# Autodesk Inventor assembly: ploter
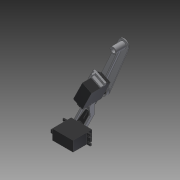
[picture p0: Inventor's stored thumbnail of the model, 180x180]
Saved by Autodesk Inventor 2013 (Build 170138000, 138)
## iProperties
Created: 2013-03-06
Part Number: ploter
Document SubType Name: Assembly
Designer: Masta
Author: Masta
## Documents named in this file (6)
- D:\work\ploter trapezowy arduino\ploter.iam
- D:\work\ploter trapezowy arduino\serwo HX12K.ipt
- D:\work\ploter trapezowy arduino\orczyk do HS12K duzy jednostronny.ipt
- D:\work\ploter trapezowy arduino\ramie1.ipt
- D:\work\ploter trapezowy arduino\ramie2.ipt
- D:\work\ploter trapezowy arduino\orczyk do SRM-102 okragly.ipt
## Components (6 placed, 5 different names)
1. serwo HX12K:1 — Insert:2
2. orczyk do HS12K duzy jednostronny:2 — Insert:2, Insert:3
3. ramie1:1 — Insert:3, Insert:4, Insert:5
4. ramie2:1 — Insert:7, Insert:8
5. serwo HX12K:2 — Insert:4, Insert:5, Insert:6
6. orczyk do SRM-102 okragly:1 — Insert:6, Insert:7, Insert:8
## Relationships (7: Insert 7)
- Insert:2: serwo HX12K:1 ↔ orczyk do HS12K duzy jednostronny:2
- Insert:3: orczyk do HS12K duzy jednostronny:2 ↔ ramie1:1
- Insert:4: ramie1:1 ↔ serwo HX12K:2
- Insert:5: ramie1:1 ↔ serwo HX12K:2
- Insert:6: serwo HX12K:2 ↔ orczyk do SRM-102 okragly:1
- Insert:7: ramie2:1 ↔ orczyk do SRM-102 okragly:1
- Insert:8: ramie2:1 ↔ orczyk do SRM-102 okragly:1
